# Autodesk Inventor assembly: Rocket
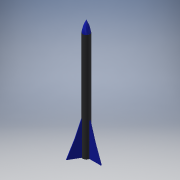
[picture p0: Inventor's stored thumbnail of the model, 180x180]
Saved by Autodesk Inventor 2018 (Build 220112000, 112)
## iProperties
Created: 2017-10-09
Part Number: Rocket
Document SubType Name: Assembly
Designer: Intel
Author: Intel
## Documents named in this file (4)
- C:\Users\Intel\Documents\Inventor\Rocket Partz\Rocket.iam
- C:\Users\Intel\Documents\Inventor\Rocket Partz\NoseCone.ipt
- C:\Users\Intel\Documents\Inventor\Rocket Partz\Body.ipt
- C:\Users\Intel\Documents\Inventor\Rocket Partz\Fin.ipt
## Components (5 placed, 3 different names)
1. NoseCone:1 — Mate:1, Mate:2
2. Body:1 — Mate:1, Mate:2, Mate:3, Flush:1, Tangent:1, Mate:4, Flush:2, Tangent:2, Mate:5, Flush:3, Tangent:3
3. Fin:1 — Mate:3, Flush:1, Tangent:1
4. Fin:2 — Mate:4, Flush:2, Tangent:2
5. Fin:3 — Mate:5, Flush:3, Tangent:3
## Relationships (11: Mate 5, Flush 3, Tangent 3)
- Mate:1: NoseCone:1 ↔ Body:1
- Mate:2: NoseCone:1 ↔ Body:1
- Mate:3: Body:1 ↔ Fin:1
- Flush:1: Body:1 ↔ Fin:1
- Tangent:1: Body:1 ↔ Fin:1
- Mate:4: Body:1 ↔ Fin:2
- Flush:2: Body:1 ↔ Fin:2
- Tangent:2: Body:1 ↔ Fin:2
- Mate:5: Body:1 ↔ Fin:3
- Flush:3: Body:1 ↔ Fin:3
- Tangent:3: Body:1 ↔ Fin:3
